# Autodesk Inventor assembly: mg996r_bottom
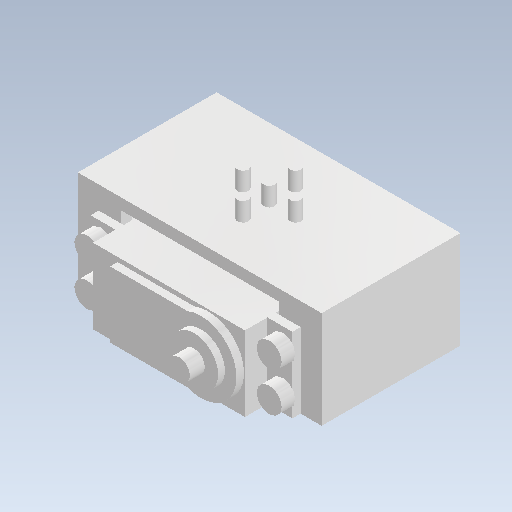
[picture p0: Inventor's stored thumbnail of the model, 512x512]
Saved by Autodesk Inventor 2021.4 (Build 254397000, 397)
## iProperties
Created: 2022-07-25
Part Number: mg996r_bottom
Document SubType Name: Assembly
Designer: isamu
Author: isamu
## Documents named in this file (3)
- D:\personal_projects\robot\inventor\2021_matlab_compat _v2\motor_with_frames\mg996r_bottom.iam
- D:\personal_projects\robot\inventor\2021_matlab_compat _v2\servo_frames\servo_bottom_frame_with_nuts.iam
- D:\personal_projects\robot\inventor\2021_matlab_compat _v2\motor\mg996r_motor_with_screws.iam
## Components (2 placed, 2 different names)
1. servo_bottom_frame_with_nuts:1 [sub-assembly] — Mate:1, Mate:2, Mate:3
2. mg996r_motor_with_screws:1 [sub-assembly] — Mate:1, Mate:2, Mate:3
## Relationships (3: Mate 3)
- Mate:1: servo_bottom_frame_with_nuts:1 ↔ mg996r_motor_with_screws:1
- Mate:2: servo_bottom_frame_with_nuts:1 ↔ mg996r_motor_with_screws:1
- Mate:3: servo_bottom_frame_with_nuts:1 ↔ mg996r_motor_with_screws:1
